# Autodesk Inventor assembly: S2_Work_Area_500
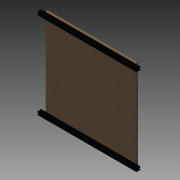
[picture p0: Inventor's stored thumbnail of the model, 180x180]
Saved by Autodesk Inventor 2014 (Build 180170000, 170)
## iProperties
Created: 2013-09-18
Part Number: S2_Work_Area_500
Document SubType Name: Assembly
Designer: Edward
Author: Edward
## Documents named in this file (6)
- C:\Users\Edward\Documents\GitHub\Shapeoko_2\S2_Work_Area_500.iam
- C:\Users\Edward\Documents\GitHub\Shapeoko_2\25286-02.ipt
- C:\Users\Edward\Documents\GitHub\Shapeoko_2\25287-02.ipt
- C:\Users\Edward\Documents\GitHub\Shapeoko_2\26016-01.ipt
- C:\Users\Edward\Documents\GitHub\Shapeoko_2\two_part_wastebaord_500.ipt
- C:\Users\Edward\Documents\GitHub\Shapeoko_2\26049-01_550.ipt
## Components (28 placed, 5 different names)
1. 26049-01_550:1 — Flush:4, Flush:5, Mate:4
2. 26049-01_550:2 — Flush:7, Flush:9, Flush:10
3. two_part_wastebaord_500:1 — Flush:10
4. two_part_wastebaord_500:2 — Flush:4, Flush:5, Mate:4, Flush:7, Flush:9
5. 25286-02:1
6. 25287-02:1
7. 26016-01:1
8. 25286-02:2
9. 25287-02:2
10. 26016-01:2
11. 25286-02:3
12. 25287-02:3
13. 26016-01:3
14. 25286-02:4
15. 25287-02:4
16. 26016-01:4
17. 25286-02:5
18. 25287-02:5
19. 26016-01:5
20. 25286-02:6
21. 25287-02:6
22. 26016-01:6
23. 25286-02:7
24. 25287-02:7
25. 26016-01:7
26. 25286-02:8
27. 25287-02:8
28. 26016-01:8
## Component patterns: (2 elements), (4 elements, first: 25286-02:1 + 25287-02:1 + 26016-01:1), Component Pattern 1:2 (4 elements)
## Relationships (15: Flush 8, Mate 4, Insert 2, Angle 1)
- [Flush]: 26049-01_550:1 ↔ 26049-01_550:2
- [Flush]: 26049-01_550:1 ↔ 26049-01_550:2
- [Mate]: 26049-01_550:2 ↔ two_part_wastebaord_500:1
- [Flush] (25 mm): 26049-01_550:2 ↔ two_part_wastebaord_500:1
- [Insert]: 25286-02:1 ↔ 25287-02:1
- [Insert]: two_part_wastebaord_500:2 ↔ 25287-02:1
- [Mate]: 25286-02:1 ↔ 26016-01:1
- [Mate]: 26049-01_550:1 ↔ 26016-01:1
- [Angle] (0 deg): 26049-01_550:1 ↔ 26016-01:1
- Flush:4: 26049-01_550:1 ↔ two_part_wastebaord_500:2
- Flush:5 (25 mm): 26049-01_550:1 ↔ two_part_wastebaord_500:2
- Mate:4: 26049-01_550:1 ↔ two_part_wastebaord_500:2
- Flush:7: 26049-01_550:2 ↔ two_part_wastebaord_500:2
- Flush:9: 26049-01_550:2 ↔ two_part_wastebaord_500:2
- Flush:10: 26049-01_550:2 ↔ two_part_wastebaord_500:1
## Named parameters: d150_d55_d51 = 0 mm
